# Autodesk Inventor assembly: leg
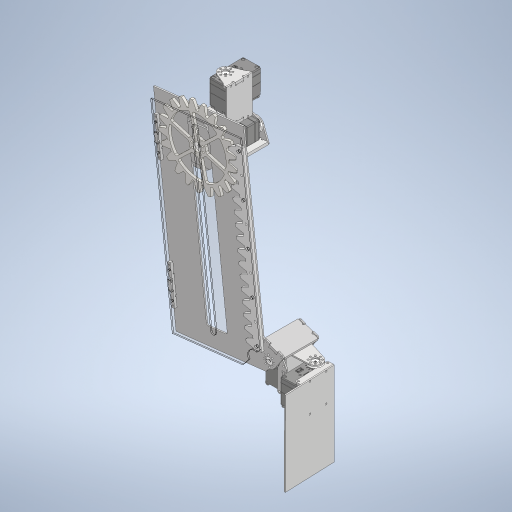
[picture p0: Inventor's stored thumbnail of the model, 512x512]
Saved by Autodesk Inventor 2024 (Build 280153000, 153)
## iProperties
Created: 2024-06-05
Part Number: leg
Document SubType Name: Assembly
Designer: right
Author: right
## Documents named in this file (23)
- C:\Users\right\OneDrive\ドキュメント\Inventor\Vixen\leg.iam
- C:\Users\right\OneDrive\ドキュメント\Inventor\Vixen\KRS2500_scale.ipt
- C:\Users\right\OneDrive\ドキュメント\Inventor\Vixen\01029_01042_LowheightServoHorn.ipt
- C:\Users\right\OneDrive\ドキュメント\Inventor\Vixen\02157_SmallDiameterHornB.ipt
- C:\Users\right\OneDrive\ドキュメント\Inventor\Vixen\02159_SmallFreeHornC\02159_SmallFreeHornC.ipt
- C:\Users\right\OneDrive\ドキュメント\Inventor\Vixen\piti_torituke.ipt
- C:\Users\right\OneDrive\ドキュメント\Inventor\Vixen\piti_entyou.ipt
- C:\Users\right\OneDrive\ドキュメント\Inventor\Vixen\free.ipt
- C:\Users\right\OneDrive\ドキュメント\Inventor\Vixen\mataroru.ipt
- C:\Users\right\OneDrive\ドキュメント\Inventor\Vixen\matarouru.ipt
- C:\Users\right\OneDrive\ドキュメント\Inventor\Vixen\freee.ipt
- C:\Users\right\OneDrive\ドキュメント\Inventor\Vixen\roruoint.ipt
- C:\Users\right\OneDrive\ドキュメント\Inventor\Vixen\SR4-500_On.ipt
- C:\Users\right\OneDrive\ドキュメント\Inventor\Vixen\leg\デザイン アクセラレータ\平歯車2.iam
- C:\Users\right\OneDrive\ドキュメント\Inventor\Vixen\sokumen.ipt
- C:\Users\right\OneDrive\ドキュメント\Inventor\Vixen\wall2.ipt
- C:\Users\right\OneDrive\ドキュメント\Inventor\Vixen\sukimaume.ipt
- C:\Users\right\OneDrive\ドキュメント\Inventor\Vixen\asikubi_ue.ipt
- C:\Users\right\OneDrive\ドキュメント\Inventor\Vixen\asikubi_2.ipt
- C:\Users\right\OneDrive\ドキュメント\Inventor\Vixen\asikubi.ipt
- C:\Users\right\OneDrive\ドキュメント\Inventor\Vixen\asikubi_setu.ipt
- C:\Users\right\OneDrive\ドキュメント\Inventor\Vixen\asiura.ipt
- C:\Users\right\OneDrive\ドキュメント\Inventor\Vixen\kabe.ipt
## Components (39 placed, 22 different names)
1. KRS2500_scale:1 — 挿入:1, フラッシュ:7, 挿入:25, 挿入:27, 角度:3, 挿入:54, 挿入:55
2. 01029_01042_LowheightServoHorn:1 — 挿入:1, 挿入:48, 挿入:49
3. KRS2500_scale:2 — 挿入:19, 挿入:22, フラッシュ:10, 挿入:33, 挿入:34
4. 02157_SmallDiameterHornB:1 — 挿入:19, 挿入:23, 挿入:24
5. 02159_SmallFreeHornC:1 — 挿入:22, 挿入:31, 挿入:32
6. piti_torituke:1 — フラッシュ:7, 挿入:23, 挿入:24, フラッシュ:8, 挿入:25, 挿入:26, 挿入:27, 挿入:28
7. piti_entyou:1 — フラッシュ:8, フラッシュ:9, 挿入:26, 挿入:28, 挿入:29, 挿入:30
8. free:1 — フラッシュ:9, 挿入:29, 挿入:30, 挿入:31, 挿入:32
9. mataroru:1 — フラッシュ:10
10. mataroru:2 — 挿入:33, 挿入:34, 挿入:39, 挿入:40
11. KRS2500_scale:3
12. 02157_SmallDiameterHornB:2 — 挿入:41, 挿入:42
13. 02159_SmallFreeHornC:2 — 挿入:43, 挿入:44
14. matarouru:1 — 挿入:39, 挿入:40, 挿入:41, 挿入:42, 角度:2, 挿入:47
15. freee:1 — 挿入:43, 挿入:44, 角度:2, 挿入:45, 挿入:46
16. roruoint:1 — 挿入:45, 挿入:46, 挿入:47
17. 平歯車:1 [sub-assembly] — 挿入:48, 挿入:49, 正接:1
18. SR4-500_On:1 — 角度:3, 正接:1, フラッシュ:11, 挿入:50, 挿入:51, フラッシュ:13
19. sokumen:1 — フラッシュ:11, 挿入:50, 挿入:51, 挿入:97, 挿入:98
20. wall2:1 — フラッシュ:13, フラッシュ:14, フラッシュ:17, 挿入:95, 挿入:96, 挿入:99, 挿入:100, 挿入:103
21. sukimaume:1 — フラッシュ:14, 挿入:54, 挿入:55
22. KRS2500_scale:4 — 挿入:59, 挿入:101, 挿入:102
23. 02157_SmallDiameterHornB:3 — 挿入:99, 挿入:100
24. 02159_SmallFreeHornC:3 — 挿入:59, 挿入:60, 挿入:61
25. free:2 — 挿入:60, 挿入:61, 挿入:88, 挿入:89
26. KRS2500_scale:5 — 挿入:104, 挿入:105, 挿入:106, 挿入:107
27. 02157_SmallDiameterHornB:4 — 挿入:76, 挿入:77
28. 02159_SmallFreeHornC:4 — 挿入:80, 挿入:81
29. asikubi_2:1 — 挿入:74, 挿入:75, 挿入:78, 挿入:79, 挿入:82, 挿入:83, 挿入:84, 挿入:85
30. asikubi:1 — 挿入:74, 挿入:75, 挿入:76, 挿入:77
31. asikubi:2 — 挿入:78, 挿入:79, 挿入:80, 挿入:81
32. asikubi_ue:1 — 挿入:82, 挿入:83
33. asikubi_ue:2 — 挿入:84, 挿入:85, 挿入:101, 挿入:102
34. piti_entyou:2 — 挿入:88, 挿入:89, 挿入:103
35. asikubi_setu:1 — 挿入:104, 挿入:105, 挿入:110
36. asikubi_setu:2 — 挿入:106, 挿入:107, 挿入:108, 挿入:109
37. asiura:1 — 挿入:108, 挿入:109, 挿入:110
38. kabe:1 — フラッシュ:17
39. kabe:2 — 挿入:95, 挿入:96, 挿入:97, 挿入:98
## Relationships (79: Insert 68, Flush 8, Angle 2, Tangent 1)
- 挿入:1 [Insert]: KRS2500_scale:1 ↔ 01029_01042_LowheightServoHorn:1
- 挿入:19 [Insert]: KRS2500_scale:2 ↔ 02157_SmallDiameterHornB:1
- 挿入:22 [Insert]: KRS2500_scale:2 ↔ 02159_SmallFreeHornC:1
- フラッシュ:7 [Flush]: KRS2500_scale:1 ↔ piti_torituke:1
- 挿入:23 [Insert]: 02157_SmallDiameterHornB:1 ↔ piti_torituke:1
- 挿入:24 [Insert]: 02157_SmallDiameterHornB:1 ↔ piti_torituke:1
- フラッシュ:8 [Flush]: piti_torituke:1 ↔ piti_entyou:1
- フラッシュ:9 [Flush]: piti_entyou:1 ↔ free:1
- 挿入:25 [Insert]: KRS2500_scale:1 ↔ piti_torituke:1
- 挿入:26 [Insert]: piti_torituke:1 ↔ piti_entyou:1
- 挿入:27 [Insert]: KRS2500_scale:1 ↔ piti_torituke:1
- 挿入:28 [Insert]: piti_torituke:1 ↔ piti_entyou:1
- 挿入:29 [Insert]: piti_entyou:1 ↔ free:1
- 挿入:30 [Insert]: piti_entyou:1 ↔ free:1
- 挿入:31 [Insert]: 02159_SmallFreeHornC:1 ↔ free:1
- 挿入:32 [Insert]: 02159_SmallFreeHornC:1 ↔ free:1
- フラッシュ:10 [Flush]: KRS2500_scale:2 ↔ mataroru:1
- 挿入:33 [Insert]: KRS2500_scale:2 ↔ mataroru:2
- 挿入:34 [Insert]: KRS2500_scale:2 ↔ mataroru:2
- [Insert]: KRS2500_scale:3 ↔ 02157_SmallDiameterHornB:2
- [Insert]: KRS2500_scale:3 ↔ 02159_SmallFreeHornC:2
- 挿入:39 [Insert]: mataroru:2 ↔ matarouru:1
- 挿入:40 [Insert]: mataroru:2 ↔ matarouru:1
- 挿入:41 [Insert]: 02157_SmallDiameterHornB:2 ↔ matarouru:1
- 挿入:42 [Insert]: 02157_SmallDiameterHornB:2 ↔ matarouru:1
- 挿入:43 [Insert]: 02159_SmallFreeHornC:2 ↔ freee:1
- 挿入:44 [Insert]: 02159_SmallFreeHornC:2 ↔ freee:1
- 角度:2 [Angle] (0 deg): matarouru:1 ↔ freee:1
- 挿入:45 [Insert]: freee:1 ↔ roruoint:1
- 挿入:46 [Insert]: freee:1 ↔ roruoint:1
- 挿入:47 [Insert]: matarouru:1 ↔ roruoint:1
- 挿入:48 [Insert]: 01029_01042_LowheightServoHorn:1 ↔ 平歯車:1
- 挿入:49 [Insert]: 01029_01042_LowheightServoHorn:1 ↔ 平歯車:1
- 角度:3 [Angle] (0 deg): KRS2500_scale:1 ↔ SR4-500_On:1
- 正接:1 [Tangent]: 平歯車:1 ↔ SR4-500_On:1
- フラッシュ:11 [Flush]: SR4-500_On:1 ↔ sokumen:1
- 挿入:50 [Insert]: SR4-500_On:1 ↔ sokumen:1
- 挿入:51 [Insert]: SR4-500_On:1 ↔ sokumen:1
- フラッシュ:13 [Flush]: SR4-500_On:1 ↔ wall2:1
- フラッシュ:14 [Flush]: wall2:1 ↔ sukimaume:1
- 挿入:54 [Insert]: KRS2500_scale:1 ↔ sukimaume:1
- 挿入:55 [Insert]: KRS2500_scale:1 ↔ sukimaume:1
- [Insert]: KRS2500_scale:4 ↔ 02157_SmallDiameterHornB:3
- 挿入:59 [Insert]: KRS2500_scale:4 ↔ 02159_SmallFreeHornC:3
- 挿入:60 [Insert]: 02159_SmallFreeHornC:3 ↔ free:2
- 挿入:61 [Insert]: 02159_SmallFreeHornC:3 ↔ free:2
- [Insert]: KRS2500_scale:5 ↔ 02157_SmallDiameterHornB:4
- [Insert]: KRS2500_scale:5 ↔ 02159_SmallFreeHornC:4
- 挿入:74 [Insert]: asikubi_2:1 ↔ asikubi:1
- 挿入:75 [Insert]: asikubi_2:1 ↔ asikubi:1
- 挿入:76 [Insert]: 02157_SmallDiameterHornB:4 ↔ asikubi:1
- 挿入:77 [Insert]: 02157_SmallDiameterHornB:4 ↔ asikubi:1
- 挿入:78 [Insert]: asikubi_2:1 ↔ asikubi:2
- 挿入:79 [Insert]: asikubi_2:1 ↔ asikubi:2
- 挿入:80 [Insert]: 02159_SmallFreeHornC:4 ↔ asikubi:2
- 挿入:81 [Insert]: 02159_SmallFreeHornC:4 ↔ asikubi:2
- 挿入:82 [Insert]: asikubi_2:1 ↔ asikubi_ue:1
- 挿入:83 [Insert]: asikubi_2:1 ↔ asikubi_ue:1
- 挿入:84 [Insert]: asikubi_2:1 ↔ asikubi_ue:2
- 挿入:85 [Insert]: asikubi_2:1 ↔ asikubi_ue:2
- 挿入:88 [Insert]: free:2 ↔ piti_entyou:2
- 挿入:89 [Insert]: free:2 ↔ piti_entyou:2
- フラッシュ:17 [Flush]: wall2:1 ↔ kabe:1
- 挿入:95 [Insert]: wall2:1 ↔ kabe:2
- 挿入:96 [Insert]: wall2:1 ↔ kabe:2
- 挿入:97 [Insert]: sokumen:1 ↔ kabe:2
- 挿入:98 [Insert]: sokumen:1 ↔ kabe:2
- 挿入:99 [Insert]: wall2:1 ↔ 02157_SmallDiameterHornB:3
- 挿入:100 [Insert]: wall2:1 ↔ 02157_SmallDiameterHornB:3
- 挿入:101 [Insert]: KRS2500_scale:4 ↔ asikubi_ue:2
- 挿入:102 [Insert]: KRS2500_scale:4 ↔ asikubi_ue:2
- 挿入:103 [Insert]: wall2:1 ↔ piti_entyou:2
- 挿入:104 [Insert]: KRS2500_scale:5 ↔ asikubi_setu:1
- 挿入:105 [Insert]: KRS2500_scale:5 ↔ asikubi_setu:1
- 挿入:106 [Insert]: KRS2500_scale:5 ↔ asikubi_setu:2
- 挿入:107 [Insert]: KRS2500_scale:5 ↔ asikubi_setu:2
- 挿入:108 [Insert]: asikubi_setu:2 ↔ asiura:1
- 挿入:109 [Insert]: asikubi_setu:2 ↔ asiura:1
- 挿入:110 [Insert]: asikubi_setu:1 ↔ asiura:1
## Named parameters: d94_d70 = 0 mm, d95_d74 = 0 mm, d135_d70 = 0 mm, d152_d135_d70 = 0 mm, d153_d138 = 0 mm
